# Autodesk Inventor assembly: upper_arm_base_with_connector
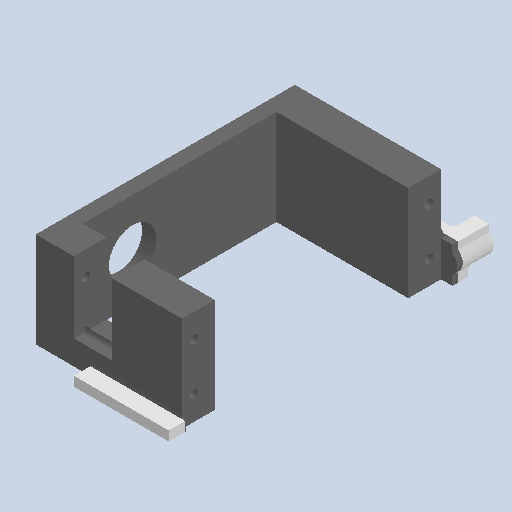
[picture p0: Inventor's stored thumbnail of the model, 512x512]
Saved by Autodesk Inventor 2024.1 (Build 281209000, 209)
## iProperties
Created: 2025-05-30
Part Number: upper_arm_base_with_connector
Document SubType Name: Assembly
Designer: hibik
Author: hibik
## Documents named in this file (3)
- C:\Users\hibik\Documents\Robomech\RESCUE\ORCA\hard\arm\upper_arm_base_with_connector.iam
- C:\Users\hibik\Documents\Robomech\RESCUE\ORCA\hard\flame_base\CORE_board_object_connector.ipt
- C:\Users\hibik\Documents\Robomech\RESCUE\ORCA\hard\arm\upper_arm_base.ipt
## Components (2 placed, 2 different names)
1. upper_arm_base:1 — フラッシュ:1, フラッシュ:2, フラッシュ:3
2. CORE_board_object_connector:1 — フラッシュ:1, フラッシュ:2, フラッシュ:3
## Relationships (3: Flush 3)
- フラッシュ:1 [Flush]: upper_arm_base:1 ↔ CORE_board_object_connector:1
- フラッシュ:2 [Flush]: upper_arm_base:1 ↔ CORE_board_object_connector:1
- フラッシュ:3 [Flush]: upper_arm_base:1 ↔ CORE_board_object_connector:1
